# Autodesk Inventor assembly: assembled-feed2
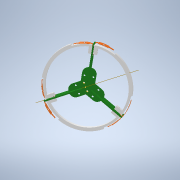
[picture p0: Inventor's stored thumbnail of the model, 180x180]
Saved by Autodesk Inventor 2021 (Build 250183000, 183)
## iProperties
Created: 2020-09-16
Part Number: assembled-feed2
Document SubType Name: Assembly
Designer: dsouthall
Author: dsouthall
## Documents named in this file (4)
- C:\Users\dsouthall\OneDrive - The University of Chicago\Hpol\Model\assembled-feed2.iam
- C:\Users\dsouthall\OneDrive - The University of Chicago\Hpol\Model\source\feedlines\tri-slot-feedlines.iam
- C:\Users\dsouthall\OneDrive - The University of Chicago\Hpol\Model\source\new_insert.ipt
- C:\Users\dsouthall\OneDrive - The University of Chicago\Hpol\Model\source\hub\tri-slot-hub.iam
## Components (7 placed, 3 different names)
1. tri-slot-feedlines:1 [sub-assembly] — Insert:1, Insert:3, Flush:1, Flush:2, Mate:1, Mate:3
2. tri-slot-feedlines:2 [sub-assembly] — Insert:4, Insert:6, Flush:2, Mate:2
3. tri-slot-feedlines:3 [sub-assembly] — Insert:2, Insert:5, Flush:1
4. new_insert:1 — Insert:5, Insert:6
5. new_insert:2 — Insert:3, Insert:4
6. new_insert:3 — Insert:1, Insert:2
7. tri-slot-hub:1 [sub-assembly] — Mate:1, Mate:2, Mate:3
## Relationships (11: Insert 6, Mate 3, Flush 2)
- Insert:1: tri-slot-feedlines:1 ↔ new_insert:3
- Insert:2: tri-slot-feedlines:3 ↔ new_insert:3
- Insert:3: tri-slot-feedlines:1 ↔ new_insert:2
- Insert:4: tri-slot-feedlines:2 ↔ new_insert:2
- Insert:5: tri-slot-feedlines:3 ↔ new_insert:1
- Insert:6: tri-slot-feedlines:2 ↔ new_insert:1
- Flush:1: tri-slot-feedlines:1 ↔ tri-slot-feedlines:3
- Flush:2: tri-slot-feedlines:1 ↔ tri-slot-feedlines:2
- Mate:1: tri-slot-feedlines:1 ↔ tri-slot-hub:1
- Mate:2: tri-slot-feedlines:2 ↔ tri-slot-hub:1
- Mate:3: tri-slot-feedlines:1 ↔ tri-slot-hub:1
